# Autodesk Inventor assembly: Soporte platos
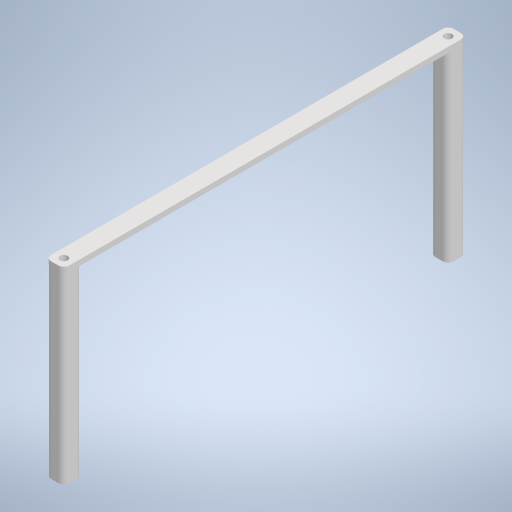
[picture p0: Inventor's stored thumbnail of the model, 512x512]
Saved by Autodesk Inventor 2024 (Build 280153000, 153)
## iProperties
Created: 2025-02-23
Part Number: Soporte platos
Document SubType Name: Assembly
Designer: sergi
Author: sergi
## Documents named in this file (3)
- C:\Users\sergi\OneDrive\Escritorio\Projects\Others\Dish Shelf\Soporte platos.iam
- C:\Users\sergi\OneDrive\Escritorio\Projects\Others\Dish Shelf\Columna.ipt
- C:\Users\sergi\OneDrive\Escritorio\Projects\Others\Dish Shelf\Tensor.ipt
## Components (3 placed, 2 different names)
1. Columna:1 — Coincidencia:3, Coincidencia:4, Nivelación:1
2. Columna:2 — Coincidencia:1, Coincidencia:2, Nivelación:2
3. Tensor:1 — Coincidencia:1, Coincidencia:2, Coincidencia:3, Coincidencia:4, Nivelación:1, Nivelación:2
## Relationships (6: Mate 4, Flush 2)
- Coincidencia:1 [Mate]: Columna:2 ↔ Tensor:1
- Coincidencia:2 [Mate]: Columna:2 ↔ Tensor:1
- Coincidencia:3 [Mate]: Columna:1 ↔ Tensor:1
- Coincidencia:4 [Mate]: Columna:1 ↔ Tensor:1
- Nivelación:1 [Flush]: Columna:1 ↔ Tensor:1
- Nivelación:2 [Flush]: Columna:2 ↔ Tensor:1
